# Autodesk Inventor assembly: INDX_000_Main
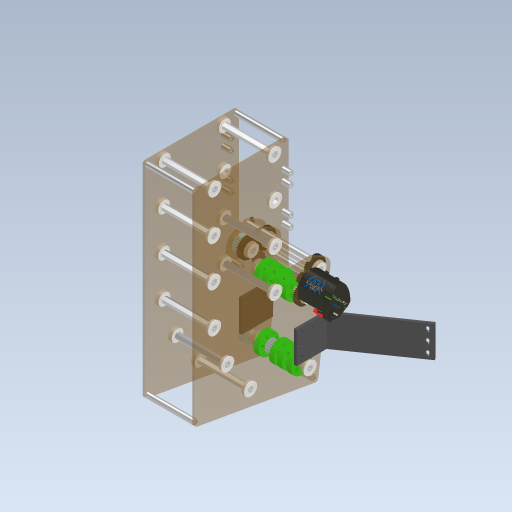
[picture p0: Inventor's stored thumbnail of the model, 512x512]
Saved by Autodesk Inventor 2024 (Build 280153000, 153)
## iProperties
Created: 2024-08-08
Part Number: INDX_000_Main
Document SubType Name: Assembly
Designer: Oscar
Author: Oscar
## Documents named in this file (22)
- C:\Users\Takum\OneDrive\Documents\GitHub\1622-2024-Summer-CAD-A-Thon\Index\INDX_000_Main.iam
- C:\Users\Takum\OneDrive\Documents\GitHub\1622-2024-Summer-CAD-A-Thon\Index\INDX_001_Plate.ipt
- C:\Users\Takum\OneDrive\Documents\GitHub\1622-2024-Summer-CAD-A-Thon\Index\INDX_002_Standoff.ipt
- C:\Users\Takum\OneDrive\Documents\GitHub\1622-2024-Summer-CAD-A-Thon\COTS Library\Motion\Bearings\COTS_WCP-0783_1.125ODHexBearing.ipt
- C:\Users\Takum\OneDrive\Documents\GitHub\1622-2024-Summer-CAD-A-Thon\COTS Library\Motors\COTS_WCP_Full_Kraken.iam
- C:\Users\Takum\OneDrive\Documents\GitHub\1622-2024-Summer-CAD-A-Thon\Index\INDX_003_OuterStandoff.ipt
- C:\Users\Takum\OneDrive\Documents\GitHub\1622-2024-Summer-CAD-A-Thon\Index\INDX_006_Funnel.ipt
- C:\Users\Takum\OneDrive\Documents\GitHub\1622-2024-Summer-CAD-A-Thon\COTS Library\Motion\Gears\Motor Gears\SplineXS\COTS_WCP-1013_14TSplineXsGear.ipt
- C:\Users\Takum\OneDrive\Documents\GitHub\1622-2024-Summer-CAD-A-Thon\COTS Library\Motion\Gears\20DP gears\Steel\0.5in hex\COTS_WCP-0174_Steel_34T20DPGear.ipt
- C:\Users\Takum\OneDrive\Documents\GitHub\1622-2024-Summer-CAD-A-Thon\Index\INDX_007_22TPulley.ipt
- C:\Users\Takum\OneDrive\Documents\GitHub\1622-2024-Summer-CAD-A-Thon\Index\INDX_008_0.5inSpacer.ipt
- C:\Users\Takum\OneDrive\Documents\GitHub\1622-2024-Summer-CAD-A-Thon\COTS Library\Motion\Wheels\Compliant Wheels\2in compliant wheels\0.500in hex bore\COTS_am-3462_2indiameter_0.500inhexbore_durometer35A_CompliantWheel.ipt
- C:\Users\Takum\OneDrive\Documents\GitHub\1622-2024-Summer-CAD-A-Thon\Index\INDX_010_5inHex.ipt
- C:\Users\Takum\OneDrive\Documents\GitHub\1622-2024-Summer-CAD-A-Thon\Index\INDX_011_SecondPlate.ipt
- C:\Users\Takum\OneDrive\Documents\GitHub\1622-2024-Summer-CAD-A-Thon\Index\INDX_012_OuterPlate.ipt
- C:\Users\Takum\OneDrive\Documents\GitHub\1622-2024-Summer-CAD-A-Thon\Index\INDX_013_ThinSpacer.ipt
- C:\Users\Takum\OneDrive\Documents\GitHub\1622-2024-Summer-CAD-A-Thon\Index\INDX_014_Outerstandoff.ipt
- C:\Users\Takum\OneDrive\Documents\GitHub\1622-2024-Summer-CAD-A-Thon\Index\INDX_009_FrontHex.ipt
- C:\Users\Takum\OneDrive\Documents\GitHub\1622-2024-Summer-CAD-A-Thon\Index\INDX_015_OuterHex.ipt
- C:\Users\Takum\OneDrive\Documents\GitHub\1622-2024-Summer-CAD-A-Thon\Index\INDX_016_BottomHex.ipt
- C:\Users\Takum\OneDrive\Documents\GitHub\1622-2024-Summer-CAD-A-Thon\COTS Library\Motion\Pulleys\HTD5M\10mm Wide\COTS_HTD5MM_9mm_16TPulley.ipt
- C:\Users\Takum\OneDrive\Documents\GitHub\1622-2024-Summer-CAD-A-Thon\Index\INDX_017_Mainhex.ipt
## Components (83 placed, 21 different names)
1. INDX_001_Plate:2 — Mate:3, Mate:5, Mate:6, Mate:9, Mate:10, Mate:12, Mate:13, Mate:14, Mate:15, Mate:16, Mate:17, Mate:18, Mate:19, Mate:20, Mate:21, Mate:22, Mate:23, Mate:24, Mate:25, Mate:26, Mate:27, Mate:28, Mate:29, Mate:30, Mate:31, Mate:54, Mate:56, Mate:57, Mate:58, Mate:59, Mate:60, Mate:61, Mate:62, Mate:63, Mate:64, Mate:65, Mate:66, Mate:67, Mate:68, Mate:69, Mate:70, Mate:79, Mate:80, Mate:81, Mate:89, Mate:162, Mate:165
2. INDX_002_Standoff:1 — Mate:9, Mate:149
3. INDX_002_Standoff:2 — Mate:6, Mate:148
4. INDX_002_Standoff:3 — Mate:10, Mate:111, Mate:150
5. INDX_002_Standoff:4 — Mate:3, Mate:5, Mate:110, Mate:112
6. COTS_WCP-0783_1.125ODHexBearing:1 — Mate:18, Mate:19
7. COTS_WCP-0783_1.125ODHexBearing:2 — Mate:16, Mate:17
8. COTS_WCP-0783_1.125ODHexBearing:3 — Mate:20, Mate:21
9. COTS_WCP-0783_1.125ODHexBearing:4 — Mate:22, Mate:23
10. COTS_WCP-0783_1.125ODHexBearing:5 — Mate:13, Mate:14
11. COTS_WCP-0783_1.125ODHexBearing:6 — Mate:12, Mate:15
12. COTS_WCP-0783_1.125ODHexBearing:7 — Mate:24, Mate:25
13. COTS_WCP-0783_1.125ODHexBearing:8 — Mate:26, Mate:27
14. COTS_WCP-0783_1.125ODHexBearing:9 — Mate:30, Mate:31
15. COTS_WCP-0783_1.125ODHexBearing:10 — Mate:28, Mate:29
16. COTS_WCP-0783_1.125ODHexBearing:11 — Mate:140, Mate:141, Mate:194, Flush:11
17. COTS_WCP-0783_1.125ODHexBearing:12 — Mate:132, Mate:133, Mate:192, Flush:9
18. COTS_WCP-0783_1.125ODHexBearing:13 — Mate:134, Mate:135
19. COTS_WCP-0783_1.125ODHexBearing:14 — Mate:146, Mate:147, Mate:189, Flush:6
20. COTS_WCP-0783_1.125ODHexBearing:15 — Mate:130, Mate:131, Mate:191, Flush:8
21. COTS_WCP-0783_1.125ODHexBearing:16 — Mate:142, Mate:143, Mate:193, Flush:10
22. COTS_WCP-0783_1.125ODHexBearing:17 — Mate:144, Mate:145, Mate:190, Flush:7
23. COTS_WCP-0783_1.125ODHexBearing:18 — Mate:96, Mate:100, Mate:102, Mate:153, Mate:154
24. COTS_WCP-0783_1.125ODHexBearing:19 — Mate:138, Mate:139, Mate:196, Flush:13
25. COTS_WCP-0783_1.125ODHexBearing:20 — Mate:113, Mate:114, Mate:195, Flush:12
26. COTS_WCP-0783_1.125ODHexBearing:21 — Mate:136, Mate:137, Mate:197, Flush:14
27. COTS_WCP_Full_Kraken:1 [sub-assembly] — Mate:54, Mate:56, Mate:89, Mate:90
28. COTS_WCP-0783_1.125ODHexBearing:22 — Mate:59, Mate:60, Mate:91, Mate:92
29. COTS_WCP-0783_1.125ODHexBearing:23 — Mate:57, Mate:58, Mate:93, Mate:94
30. COTS_WCP-0783_1.125ODHexBearing:24 — Mate:61, Mate:62, Mate:184
31. INDX_003_OuterStandoff:1 — Mate:115, Mate:116
32. INDX_003_OuterStandoff:2 — Mate:119, Mate:120
33. INDX_003_OuterStandoff:3 — Mate:63, Mate:68
34. INDX_003_OuterStandoff:4 — Mate:64, Mate:69
35. INDX_003_OuterStandoff:5 — Mate:65, Mate:70
36. INDX_003_OuterStandoff:6 — Mate:66, Mate:67
37. INDX_003_OuterStandoff:7 — Mate:117, Mate:118
38. INDX_003_OuterStandoff:8 — Mate:121, Mate:122
39. INDX_006_Funnel:1 — Mate:79, Mate:80, Mate:81
40. INDX_006_Funnel:2 — Mate:123, Mate:124, Mate:125
41. COTS_WCP-0783_1.125ODHexBearing:25 — Mate:126, Mate:127, Mate:128, Mate:129
42. COTS_WCP-0783_1.125ODHexBearing:26 — Mate:109, Flush:2, Mate:151, Mate:152
43. COTS_WCP-1013_14TSplineXsGear:1 — Mate:90
44. COTS_WCP-0174_Steel_34T20DPGear:1 — Mate:93, Mate:94, Mate:108
45. COTS_WCP-0174_Steel_34T20DPGear:2 — Mate:91, Mate:92
46. INDX_007_22TPulley:1 — Mate:159, Mate:160, Mate:172, Mate:173
47. INDX_007_22TPulley:2 — Mate:96, Mate:101, Flush:5
48. INDX_008_0.5inSpacer:1 — Mate:100, Mate:101, Mate:102, Mate:183
49. COTS_am-3462_2indiameter_0.500inhexbore_durometer35A_CompliantWheel:1 — Mate:105
50. COTS_am-3462_2indiameter_0.500inhexbore_durometer35A_CompliantWheel:2 — Mate:106, Mate:107
51. COTS_am-3462_2indiameter_0.500inhexbore_durometer35A_CompliantWheel:3 — Mate:107
52. COTS_am-3462_2indiameter_0.500inhexbore_durometer35A_CompliantWheel:4 — Mate:105, Mate:106, Mate:108
53. INDX_010_5inHex:1 — Mate:109, Flush:2
54. INDX_011_SecondPlate:1 — Mate:110, Mate:111, Mate:112, Mate:113, Mate:114, Mate:115, Mate:116, Mate:117, Mate:118, Mate:119, Mate:120, Mate:121, Mate:122, Mate:123, Mate:124, Mate:125, Mate:126, Mate:127, Mate:130, Mate:131, Mate:132, Mate:133, Mate:134, Mate:135, Mate:136, Mate:137, Mate:138, Mate:139, Mate:140, Mate:141, Mate:142, Mate:143, Mate:144, Mate:145, Mate:146, Mate:147, Mate:148, Mate:149, Mate:150, Mate:151, Mate:152, Mate:153, Mate:154, Mate:155, Mate:156, Mate:157, Mate:163, Mate:164, Mate:166, Mate:167, Mate:175, Mate:177, Mate:179
55. COTS_WCP-0174_Steel_34T20DPGear:3 — Mate:128, Mate:129, Mate:181
56. COTS_WCP-0174_Steel_34T20DPGear:4 — Mate:155, Mate:158, Mate:159, Mate:160
57. COTS_WCP-0783_1.125ODHexBearing:27 — Mate:156, Mate:157, Mate:158
58. INDX_002_Standoff:5 — Mate:162, Mate:163
59. INDX_002_Standoff:6 — Mate:164, Mate:165
60. INDX_012_OuterPlate:1 — Mate:166, Mate:167, Mate:168, Mate:169, Mate:170, Mate:171, Mate:176, Mate:178, Mate:180
61. COTS_WCP-0783_1.125ODHexBearing:28 — Mate:170, Mate:171, Mate:174, Mate:182, Flush:4
62. COTS_WCP-0783_1.125ODHexBearing:29 — Mate:168, Mate:169, Flush:3
63. INDX_013_ThinSpacer:1 — Mate:172, Mate:173, Mate:174
64. INDX_014_Outerstandoff:1 — Mate:175, Mate:176
65. INDX_014_Outerstandoff:2 — Mate:177, Mate:178
66. INDX_014_Outerstandoff:3 — Mate:179, Mate:180
67. INDX_009_FrontHex:1 — Mate:181, Flush:3
68. INDX_015_OuterHex:1 — Mate:182, Flush:4
69. INDX_016_BottomHex:1 — Mate:183, Flush:5
70. COTS_am-3462_2indiameter_0.500inhexbore_durometer35A_CompliantWheel:5 — Mate:184, Mate:185, Mate:186
71. COTS_am-3462_2indiameter_0.500inhexbore_durometer35A_CompliantWheel:6 — Mate:185
72. COTS_am-3462_2indiameter_0.500inhexbore_durometer35A_CompliantWheel:7 — Mate:186, Mate:187, Mate:188
73. COTS_am-3462_2indiameter_0.500inhexbore_durometer35A_CompliantWheel:8 — Mate:187
74. COTS_HTD5MM_9mm_16TPulley:1 — Mate:188
75. INDX_017_Mainhex:1 — Mate:190, Flush:7
76. INDX_017_Mainhex:2 — Mate:189, Flush:6
77. INDX_017_Mainhex:3 — Mate:192, Flush:9
78. INDX_017_Mainhex:4 — Mate:193, Flush:10
79. INDX_017_Mainhex:5 — Mate:191, Flush:8
80. INDX_017_Mainhex:6 — Mate:194, Flush:11
81. INDX_017_Mainhex:7 — Mate:195, Flush:12
82. INDX_017_Mainhex:8 — Mate:196, Flush:13
83. INDX_017_Mainhex:9 — Mate:197, Flush:14
## Relationships (159: Mate 146, Flush 13)
- Mate:3: INDX_001_Plate:2 ↔ INDX_002_Standoff:4
- Mate:5: INDX_001_Plate:2 ↔ INDX_002_Standoff:4
- Mate:6: INDX_001_Plate:2 ↔ INDX_002_Standoff:2
- Mate:9: INDX_001_Plate:2 ↔ INDX_002_Standoff:1
- Mate:10: INDX_001_Plate:2 ↔ INDX_002_Standoff:3
- Mate:12: INDX_001_Plate:2 ↔ COTS_WCP-0783_1.125ODHexBearing:6
- Mate:13: INDX_001_Plate:2 ↔ COTS_WCP-0783_1.125ODHexBearing:5
- Mate:14: INDX_001_Plate:2 ↔ COTS_WCP-0783_1.125ODHexBearing:5
- Mate:15: INDX_001_Plate:2 ↔ COTS_WCP-0783_1.125ODHexBearing:6
- Mate:16: INDX_001_Plate:2 ↔ COTS_WCP-0783_1.125ODHexBearing:2
- Mate:17: INDX_001_Plate:2 ↔ COTS_WCP-0783_1.125ODHexBearing:2
- Mate:18: INDX_001_Plate:2 ↔ COTS_WCP-0783_1.125ODHexBearing:1
- Mate:19: INDX_001_Plate:2 ↔ COTS_WCP-0783_1.125ODHexBearing:1
- Mate:20: INDX_001_Plate:2 ↔ COTS_WCP-0783_1.125ODHexBearing:3
- Mate:21: INDX_001_Plate:2 ↔ COTS_WCP-0783_1.125ODHexBearing:3
- Mate:22: INDX_001_Plate:2 ↔ COTS_WCP-0783_1.125ODHexBearing:4
- Mate:23: INDX_001_Plate:2 ↔ COTS_WCP-0783_1.125ODHexBearing:4
- Mate:24: INDX_001_Plate:2 ↔ COTS_WCP-0783_1.125ODHexBearing:7
- Mate:25: INDX_001_Plate:2 ↔ COTS_WCP-0783_1.125ODHexBearing:7
- Mate:26: INDX_001_Plate:2 ↔ COTS_WCP-0783_1.125ODHexBearing:8
- Mate:27: INDX_001_Plate:2 ↔ COTS_WCP-0783_1.125ODHexBearing:8
- Mate:28: INDX_001_Plate:2 ↔ COTS_WCP-0783_1.125ODHexBearing:10
- Mate:29: INDX_001_Plate:2 ↔ COTS_WCP-0783_1.125ODHexBearing:10
- Mate:30: INDX_001_Plate:2 ↔ COTS_WCP-0783_1.125ODHexBearing:9
- Mate:31: INDX_001_Plate:2 ↔ COTS_WCP-0783_1.125ODHexBearing:9
- Mate:54: INDX_001_Plate:2 ↔ COTS_WCP_Full_Kraken:1
- Mate:56: INDX_001_Plate:2 ↔ COTS_WCP_Full_Kraken:1
- Mate:57: INDX_001_Plate:2 ↔ COTS_WCP-0783_1.125ODHexBearing:23
- Mate:58: INDX_001_Plate:2 ↔ COTS_WCP-0783_1.125ODHexBearing:23
- Mate:59: INDX_001_Plate:2 ↔ COTS_WCP-0783_1.125ODHexBearing:22
- Mate:60: INDX_001_Plate:2 ↔ COTS_WCP-0783_1.125ODHexBearing:22
- Mate:61: INDX_001_Plate:2 ↔ COTS_WCP-0783_1.125ODHexBearing:24
- Mate:62: INDX_001_Plate:2 ↔ COTS_WCP-0783_1.125ODHexBearing:24
- Mate:63: INDX_001_Plate:2 ↔ INDX_003_OuterStandoff:3
- Mate:64: INDX_001_Plate:2 ↔ INDX_003_OuterStandoff:4
- Mate:65: INDX_001_Plate:2 ↔ INDX_003_OuterStandoff:5
- Mate:66: INDX_001_Plate:2 ↔ INDX_003_OuterStandoff:6
- Mate:67: INDX_001_Plate:2 ↔ INDX_003_OuterStandoff:6
- Mate:68: INDX_001_Plate:2 ↔ INDX_003_OuterStandoff:3
- Mate:69: INDX_001_Plate:2 ↔ INDX_003_OuterStandoff:4
- Mate:70: INDX_001_Plate:2 ↔ INDX_003_OuterStandoff:5
- Mate:79: INDX_001_Plate:2 ↔ INDX_006_Funnel:1
- Mate:80: INDX_001_Plate:2 ↔ INDX_006_Funnel:1
- Mate:81: INDX_001_Plate:2 ↔ INDX_006_Funnel:1
- Mate:89: INDX_001_Plate:2 ↔ COTS_WCP_Full_Kraken:1
- Mate:90: COTS_WCP_Full_Kraken:1 ↔ COTS_WCP-1013_14TSplineXsGear:1
- Mate:91: COTS_WCP-0783_1.125ODHexBearing:22 ↔ COTS_WCP-0174_Steel_34T20DPGear:2
- Mate:92: COTS_WCP-0783_1.125ODHexBearing:22 ↔ COTS_WCP-0174_Steel_34T20DPGear:2
- Mate:93: COTS_WCP-0783_1.125ODHexBearing:23 ↔ COTS_WCP-0174_Steel_34T20DPGear:1
- Mate:94: COTS_WCP-0783_1.125ODHexBearing:23 ↔ COTS_WCP-0174_Steel_34T20DPGear:1
- Mate:96: COTS_WCP-0783_1.125ODHexBearing:18 ↔ INDX_007_22TPulley:2
- Mate:100: COTS_WCP-0783_1.125ODHexBearing:18 ↔ INDX_008_0.5inSpacer:1
- Mate:101: INDX_007_22TPulley:2 ↔ INDX_008_0.5inSpacer:1
- Mate:102: COTS_WCP-0783_1.125ODHexBearing:18 ↔ INDX_008_0.5inSpacer:1
- Mate:105: COTS_am-3462_2indiameter_0.500inhexbore_durometer35A_CompliantWheel:1 ↔ COTS_am-3462_2indiameter_0.500inhexbore_durometer35A_CompliantWheel:4
- Mate:106: COTS_am-3462_2indiameter_0.500inhexbore_durometer35A_CompliantWheel:2 ↔ COTS_am-3462_2indiameter_0.500inhexbore_durometer35A_CompliantWheel:4
- Mate:107: COTS_am-3462_2indiameter_0.500inhexbore_durometer35A_CompliantWheel:2 ↔ COTS_am-3462_2indiameter_0.500inhexbore_durometer35A_CompliantWheel:3
- Mate:108: COTS_WCP-0174_Steel_34T20DPGear:1 ↔ COTS_am-3462_2indiameter_0.500inhexbore_durometer35A_CompliantWheel:4
- Mate:109: COTS_WCP-0783_1.125ODHexBearing:26 ↔ INDX_010_5inHex:1
- Flush:2: COTS_WCP-0783_1.125ODHexBearing:26 ↔ INDX_010_5inHex:1
- Mate:110: INDX_002_Standoff:4 ↔ INDX_011_SecondPlate:1
- Mate:111: INDX_002_Standoff:3 ↔ INDX_011_SecondPlate:1
- Mate:112: INDX_002_Standoff:4 ↔ INDX_011_SecondPlate:1
- Mate:113: COTS_WCP-0783_1.125ODHexBearing:20 ↔ INDX_011_SecondPlate:1
- Mate:114: COTS_WCP-0783_1.125ODHexBearing:20 ↔ INDX_011_SecondPlate:1
- Mate:115: INDX_003_OuterStandoff:1 ↔ INDX_011_SecondPlate:1
- Mate:116: INDX_003_OuterStandoff:1 ↔ INDX_011_SecondPlate:1
- Mate:117: INDX_003_OuterStandoff:7 ↔ INDX_011_SecondPlate:1
- Mate:118: INDX_003_OuterStandoff:7 ↔ INDX_011_SecondPlate:1
- Mate:119: INDX_003_OuterStandoff:2 ↔ INDX_011_SecondPlate:1
- Mate:120: INDX_003_OuterStandoff:2 ↔ INDX_011_SecondPlate:1
- Mate:121: INDX_003_OuterStandoff:8 ↔ INDX_011_SecondPlate:1
- Mate:122: INDX_003_OuterStandoff:8 ↔ INDX_011_SecondPlate:1
- Mate:123: INDX_006_Funnel:2 ↔ INDX_011_SecondPlate:1
- Mate:124: INDX_006_Funnel:2 ↔ INDX_011_SecondPlate:1
- Mate:125: INDX_006_Funnel:2 ↔ INDX_011_SecondPlate:1
- Mate:126: COTS_WCP-0783_1.125ODHexBearing:25 ↔ INDX_011_SecondPlate:1
- Mate:127: COTS_WCP-0783_1.125ODHexBearing:25 ↔ INDX_011_SecondPlate:1
- Mate:128: COTS_WCP-0783_1.125ODHexBearing:25 ↔ COTS_WCP-0174_Steel_34T20DPGear:3
- Mate:129: COTS_WCP-0783_1.125ODHexBearing:25 ↔ COTS_WCP-0174_Steel_34T20DPGear:3
- Mate:130: COTS_WCP-0783_1.125ODHexBearing:15 ↔ INDX_011_SecondPlate:1
- Mate:131: COTS_WCP-0783_1.125ODHexBearing:15 ↔ INDX_011_SecondPlate:1
- Mate:132: COTS_WCP-0783_1.125ODHexBearing:12 ↔ INDX_011_SecondPlate:1
- Mate:133: COTS_WCP-0783_1.125ODHexBearing:12 ↔ INDX_011_SecondPlate:1
- Mate:134: COTS_WCP-0783_1.125ODHexBearing:13 ↔ INDX_011_SecondPlate:1
- Mate:135: COTS_WCP-0783_1.125ODHexBearing:13 ↔ INDX_011_SecondPlate:1
- Mate:136: COTS_WCP-0783_1.125ODHexBearing:21 ↔ INDX_011_SecondPlate:1
- Mate:137: COTS_WCP-0783_1.125ODHexBearing:21 ↔ INDX_011_SecondPlate:1
- Mate:138: COTS_WCP-0783_1.125ODHexBearing:19 ↔ INDX_011_SecondPlate:1
- Mate:139: COTS_WCP-0783_1.125ODHexBearing:19 ↔ INDX_011_SecondPlate:1
- Mate:140: COTS_WCP-0783_1.125ODHexBearing:11 ↔ INDX_011_SecondPlate:1
- Mate:141: COTS_WCP-0783_1.125ODHexBearing:11 ↔ INDX_011_SecondPlate:1
- Mate:142: COTS_WCP-0783_1.125ODHexBearing:16 ↔ INDX_011_SecondPlate:1
- Mate:143: COTS_WCP-0783_1.125ODHexBearing:16 ↔ INDX_011_SecondPlate:1
- Mate:144: COTS_WCP-0783_1.125ODHexBearing:17 ↔ INDX_011_SecondPlate:1
- Mate:145: COTS_WCP-0783_1.125ODHexBearing:17 ↔ INDX_011_SecondPlate:1
- Mate:146: COTS_WCP-0783_1.125ODHexBearing:14 ↔ INDX_011_SecondPlate:1
- Mate:147: COTS_WCP-0783_1.125ODHexBearing:14 ↔ INDX_011_SecondPlate:1
- Mate:148: INDX_002_Standoff:2 ↔ INDX_011_SecondPlate:1
- Mate:149: INDX_002_Standoff:1 ↔ INDX_011_SecondPlate:1
- Mate:150: INDX_002_Standoff:3 ↔ INDX_011_SecondPlate:1
- Mate:151: COTS_WCP-0783_1.125ODHexBearing:26 ↔ INDX_011_SecondPlate:1
- Mate:152: COTS_WCP-0783_1.125ODHexBearing:26 ↔ INDX_011_SecondPlate:1
- Mate:153: COTS_WCP-0783_1.125ODHexBearing:18 ↔ INDX_011_SecondPlate:1
- Mate:154: COTS_WCP-0783_1.125ODHexBearing:18 ↔ INDX_011_SecondPlate:1
- Mate:155: INDX_011_SecondPlate:1 ↔ COTS_WCP-0174_Steel_34T20DPGear:4
- Mate:156: INDX_011_SecondPlate:1 ↔ COTS_WCP-0783_1.125ODHexBearing:27
- Mate:157: INDX_011_SecondPlate:1 ↔ COTS_WCP-0783_1.125ODHexBearing:27
- Mate:158: COTS_WCP-0174_Steel_34T20DPGear:4 ↔ COTS_WCP-0783_1.125ODHexBearing:27
- Mate:159: INDX_007_22TPulley:1 ↔ COTS_WCP-0174_Steel_34T20DPGear:4
- Mate:160: INDX_007_22TPulley:1 ↔ COTS_WCP-0174_Steel_34T20DPGear:4
- Mate:162: INDX_001_Plate:2 ↔ INDX_002_Standoff:5
- Mate:163: INDX_011_SecondPlate:1 ↔ INDX_002_Standoff:5
- Mate:164: INDX_011_SecondPlate:1 ↔ INDX_002_Standoff:6
- Mate:165: INDX_001_Plate:2 ↔ INDX_002_Standoff:6
- Mate:166: INDX_011_SecondPlate:1 ↔ INDX_012_OuterPlate:1
- Mate:167: INDX_011_SecondPlate:1 ↔ INDX_012_OuterPlate:1
- Mate:168: INDX_012_OuterPlate:1 ↔ COTS_WCP-0783_1.125ODHexBearing:29
- Mate:169: INDX_012_OuterPlate:1 ↔ COTS_WCP-0783_1.125ODHexBearing:29
- Mate:170: INDX_012_OuterPlate:1 ↔ COTS_WCP-0783_1.125ODHexBearing:28
- Mate:171: INDX_012_OuterPlate:1 ↔ COTS_WCP-0783_1.125ODHexBearing:28
- Mate:172: INDX_007_22TPulley:1 ↔ INDX_013_ThinSpacer:1
- Mate:173: INDX_007_22TPulley:1 ↔ INDX_013_ThinSpacer:1
- Mate:174: COTS_WCP-0783_1.125ODHexBearing:28 ↔ INDX_013_ThinSpacer:1
- Mate:175: INDX_011_SecondPlate:1 ↔ INDX_014_Outerstandoff:1
- Mate:176: INDX_012_OuterPlate:1 ↔ INDX_014_Outerstandoff:1
- Mate:177: INDX_011_SecondPlate:1 ↔ INDX_014_Outerstandoff:2
- Mate:178: INDX_012_OuterPlate:1 ↔ INDX_014_Outerstandoff:2
- Mate:179: INDX_011_SecondPlate:1 ↔ INDX_014_Outerstandoff:3
- Mate:180: INDX_012_OuterPlate:1 ↔ INDX_014_Outerstandoff:3
- Mate:181: COTS_WCP-0174_Steel_34T20DPGear:3 ↔ INDX_009_FrontHex:1
- Flush:3: COTS_WCP-0783_1.125ODHexBearing:29 ↔ INDX_009_FrontHex:1
- Mate:182: COTS_WCP-0783_1.125ODHexBearing:28 ↔ INDX_015_OuterHex:1
- Flush:4: COTS_WCP-0783_1.125ODHexBearing:28 ↔ INDX_015_OuterHex:1
- Mate:183: INDX_008_0.5inSpacer:1 ↔ INDX_016_BottomHex:1
- Flush:5: INDX_007_22TPulley:2 ↔ INDX_016_BottomHex:1
- Mate:184: COTS_WCP-0783_1.125ODHexBearing:24 ↔ COTS_am-3462_2indiameter_0.500inhexbore_durometer35A_CompliantWheel:5
- Mate:185: COTS_am-3462_2indiameter_0.500inhexbore_durometer35A_CompliantWheel:5 ↔ COTS_am-3462_2indiameter_0.500inhexbore_durometer35A_CompliantWheel:6
- Mate:186: COTS_am-3462_2indiameter_0.500inhexbore_durometer35A_CompliantWheel:5 ↔ COTS_am-3462_2indiameter_0.500inhexbore_durometer35A_CompliantWheel:7
- Mate:187: COTS_am-3462_2indiameter_0.500inhexbore_durometer35A_CompliantWheel:7 ↔ COTS_am-3462_2indiameter_0.500inhexbore_durometer35A_CompliantWheel:8
- Mate:188: COTS_am-3462_2indiameter_0.500inhexbore_durometer35A_CompliantWheel:7 ↔ COTS_HTD5MM_9mm_16TPulley:1
- Mate:189: COTS_WCP-0783_1.125ODHexBearing:14 ↔ INDX_017_Mainhex:2
- Flush:6: COTS_WCP-0783_1.125ODHexBearing:14 ↔ INDX_017_Mainhex:2
- Mate:190: COTS_WCP-0783_1.125ODHexBearing:17 ↔ INDX_017_Mainhex:1
- Flush:7: COTS_WCP-0783_1.125ODHexBearing:17 ↔ INDX_017_Mainhex:1
- Mate:191: COTS_WCP-0783_1.125ODHexBearing:15 ↔ INDX_017_Mainhex:5
- Flush:8: COTS_WCP-0783_1.125ODHexBearing:15 ↔ INDX_017_Mainhex:5
- Mate:192: COTS_WCP-0783_1.125ODHexBearing:12 ↔ INDX_017_Mainhex:3
- Flush:9: COTS_WCP-0783_1.125ODHexBearing:12 ↔ INDX_017_Mainhex:3
- Mate:193: COTS_WCP-0783_1.125ODHexBearing:16 ↔ INDX_017_Mainhex:4
- Flush:10: COTS_WCP-0783_1.125ODHexBearing:16 ↔ INDX_017_Mainhex:4
- Mate:194: COTS_WCP-0783_1.125ODHexBearing:11 ↔ INDX_017_Mainhex:6
- Flush:11: COTS_WCP-0783_1.125ODHexBearing:11 ↔ INDX_017_Mainhex:6
- Mate:195: COTS_WCP-0783_1.125ODHexBearing:20 ↔ INDX_017_Mainhex:7
- Flush:12: COTS_WCP-0783_1.125ODHexBearing:20 ↔ INDX_017_Mainhex:7
- Mate:196: COTS_WCP-0783_1.125ODHexBearing:19 ↔ INDX_017_Mainhex:8
- Flush:13: COTS_WCP-0783_1.125ODHexBearing:19 ↔ INDX_017_Mainhex:8
- Mate:197: COTS_WCP-0783_1.125ODHexBearing:21 ↔ INDX_017_Mainhex:9
- Flush:14: COTS_WCP-0783_1.125ODHexBearing:21 ↔ INDX_017_Mainhex:9
